# Autodesk Inventor assembly: Joint Housing Bottom
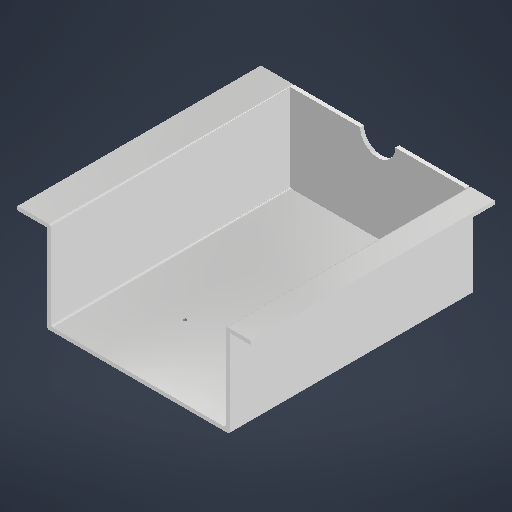
[picture p0: Inventor's stored thumbnail of the model, 512x512]
Saved by Autodesk Inventor 2026.3 (Build 303398000, 398)
## iProperties
Created: 2026-07-26
Part Number: Joint Housing Bottom
Document SubType Name: Assembly
Designer: matot
Author: matot
## Documents named in this file (3)
- C:\Users\matot\OneDrive - Stellenbosch University\2026\MechatronicsProject478\Building the joint\Joint Assembly\Joint Housing Bottom.iam
- C:\Users\matot\OneDrive - Stellenbosch University\2026\MechatronicsProject478\Building the joint\Joint Assembly\Lower joint housing.ipt
- C:\Users\matot\OneDrive - Stellenbosch University\2026\MechatronicsProject478\Building the joint\Joint Assembly\Joint housing cover.ipt
## Components (2 placed, 2 different names)
1. Lower joint housing:1 — Flush:1, Mate:2, Mate:3
2. Joint housing cover:1 — Flush:1, Mate:2, Mate:3
## Relationships (3: Mate 2, Flush 1)
- Flush:1: Lower joint housing:1 ↔ Joint housing cover:1
- Mate:2: Lower joint housing:1 ↔ Joint housing cover:1
- Mate:3: Lower joint housing:1 ↔ Joint housing cover:1
